# Autodesk Inventor assembly: vexFrisbeeShooter10
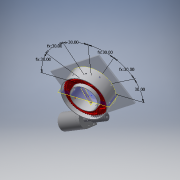
[picture p0: Inventor's stored thumbnail of the model, 180x180]
Saved by Autodesk Inventor 2016 SP1 (Build 200210100, 210)
## iProperties
Created: 2015-11-02
Part Number: vexFrisbeeShooter10
Document SubType Name: Assembly
Designer: steele
Author: steele
## Documents named in this file (7)
- C:\snobotics\CAD-Development\robSteele\FRC 2013 Ultimate Ascent\vexFrisbeeShooter10.iam
- C:\snobotics\CAD-Development\robSteele\FRC 2013 Ultimate Ascent\vexFrisbeeShooter10\Design Accelerator\Worm Gears1.iam
- C:\snobotics\CAD-MfgResources\VexRobotics\Motors\Vex Mini Cim 217-3371.ipt
- C:\snobotics\CAD-MfgResources\Andy-Mark\MotorMounts\AM 2488 CIM bracket.ipt
- C:\snobotics\CAD-Development\robSteele\FRC 2013 Ultimate Ascent\LexanBasePlate.ipt
- C:\snobotics\CAD-Development\robSteele\FRC 2013 Ultimate Ascent\vexInnerFrisbeeHopper.ipt
- C:\snobotics\CAD-Development\robSteele\FRC 2013 Ultimate Ascent\vexOuterFrisbeeHopper.ipt
## Components (6 placed, 6 different names)
1. Worm Gears:1 [sub-assembly] — Insert:1, Insert:3
2. Vex Mini Cim 217-3371:1 — Insert:1, Insert:2
3. AM 2488 CIM bracket:1 — Insert:2
4. LexanBasePlate:1 — Insert:3, Insert:4, Insert:5
5. vexInnerFrisbeeHopper:1 — Insert:4
6. vexOuterFrisbeeHopper:1 — Insert:5
## Relationships (5: Insert 5)
- Insert:1: Worm Gears:1 ↔ Vex Mini Cim 217-3371:1
- Insert:2: Vex Mini Cim 217-3371:1 ↔ AM 2488 CIM bracket:1
- Insert:3 (33.3502 mm): Worm Gears:1 ↔ LexanBasePlate:1
- Insert:4: LexanBasePlate:1 ↔ vexInnerFrisbeeHopper:1
- Insert:5: LexanBasePlate:1 ↔ vexOuterFrisbeeHopper:1
